# Autodesk Inventor assembly: M178-PHTM-3000-01
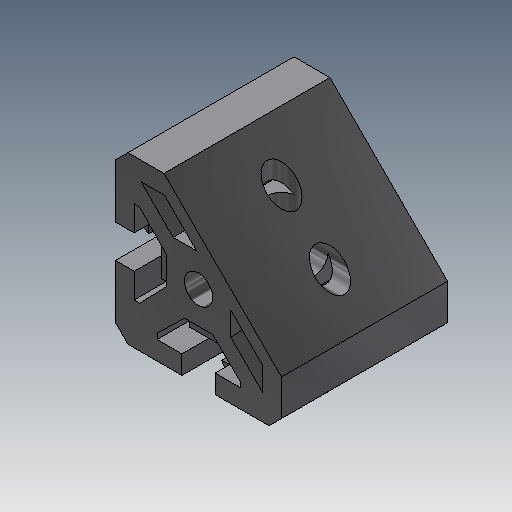
[picture p0: Inventor's stored thumbnail of the model, 512x512]
Saved by Autodesk Inventor 2018.3 (Build 223284000, 284)
## iProperties
Created: 2004-11-23
Part Number: M178-PHTM-3000-01
Document SubType Name: Assembly
Designer: Autodesk, Inc.
Manufacturer: Standard
Standards Organization: Custom
Description: PHANTOM, CORNER BRACKET 1
Mass: 135.083 g
Surface Area: 199.405 cm^2
Volume: 36.5913 cm^3
Density: 3.69168 g/cm^3
CAGE: 1LJX3
Dept. ID: Product Design
Description #2: ---
Finish #1: ---
Finish #2: ---
Material ID: ---
Project Number: ---
Author: Autodesk, Inc.
## Documents named in this file (6)
- C:\AVAInvAPI\Workspace\Test Station\Components\21-135 Corner Phantom.iam
- C:\AVAInvAPI\Workspace\Test Station\Components\21-135.ipt
- C:\AVAInvAPI\Workspace\Test Station\Components\20-028.iam
- C:\AVAInvAPI\Workspace\Test Station\Components\20-058.ipt
- C:\Users\kelleyb.ADS\Desktop\Samples MIGRATED 2009 224 RTM_1\Standard Parts\Test Station Content\Corners, Gussets, and Mounting Plates\21-XXX Corner Elements.ipt
- C:\Users\kelleyb.ADS\Desktop\Samples MIGRATED 2009 224 RTM_1\Standard Parts\Test Station Content\Fastners\20-XXX TSlot Nuts.ipt
## Components (5 placed, 3 different names)
1. 21-135:1 — Mate:3, Mate:4, Angle:2, Mate:7, Angle:4
2. 20-028:2 [sub-assembly] — Mate:3, Mate:4, Angle:2, Mate:6
3. 20-058:2 — Mate:6, Mate:7, Angle:4
4. 20-028:3 [sub-assembly]
5. 20-058:3
## Component patterns: (2 elements, first: 20-028:2 + 20-058:2)
## Relationships (6: Mate 4, Angle 2)
- Mate:3: 21-135:1 ↔ 20-028:2
- Mate:4: 21-135:1 ↔ 20-028:2
- Angle:2 (0 deg): 21-135:1 ↔ 20-028:2
- Mate:6: 20-028:2 ↔ 20-058:2
- Mate:7 (4.5 mm): 21-135:1 ↔ 20-058:2
- Angle:4 (0 deg): 21-135:1 ↔ 20-058:2
